# Autodesk Inventor assembly: Pin Header 20x2 TH Pitch 2.54mm v1
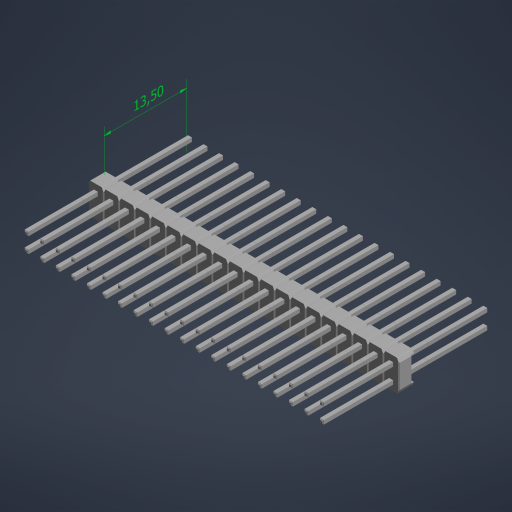
[picture p0: Inventor's stored thumbnail of the model, 512x512]
Saved by Autodesk Inventor 2023 (Build 270158030, 158C)
## iProperties
Created: 2018-05-25
Part Number: Pin Header 20x2 TH Pitch 2.54mm v1
Document SubType Name: Assembly
Designer: Administrator
Title: Pin Header 20x2 TH Pitch 2.54mm v1
Author: Administrator
## Documents named in this file (4)
- C:\Users\norbe\Repozytoria\NormalMapScanner\3D_modeling\construction\parts\external_parts\raspberry_goldpins_2x40\Pin Header 20x2 TH Pitch 2.54mm v1.iam
- C:\Users\norbe\Repozytoria\NormalMapScanner\3D_modeling\construction\parts\external_parts\raspberry_goldpins_2x40\pins.ipt
- C:\Users\norbe\Repozytoria\NormalMapScanner\3D_modeling\construction\parts\external_parts\raspberry_goldpins_2x40\spacers.iam
- C:\Users\norbe\Repozytoria\NormalMapScanner\3D_modeling\construction\parts\external_parts\raspberry_goldpins_2x40\pins_CPY.ipt
## Components (4 placed, 3 different names)
1. pins:1 — Mate:1, Mate:2, Mate:3, Flush:1, Flush:2, Flush:3, Mate:4
2. spacers:1 [sub-assembly] — Mate:1, Mate:2, Mate:3
3. pins_CPY:1 — Flush:1, Flush:2, Flush:3, Mate:4, Flush:4, Flush:5, Mate:5
4. pins_CPY:2 — Flush:4, Flush:5, Mate:5
## Relationships (10: Mate 5, Flush 5)
- Mate:1: pins:1 ↔ spacers:1
- Mate:2: pins:1 ↔ spacers:1
- Mate:3 (-14 mm): pins:1 ↔ spacers:1
- Flush:1: pins:1 ↔ pins_CPY:1
- Flush:2: pins:1 ↔ pins_CPY:1
- Flush:3: pins:1 ↔ pins_CPY:1
- Mate:4 (-1 mm): pins:1 ↔ pins_CPY:1
- Flush:4: pins_CPY:1 ↔ pins_CPY:2
- Flush:5: pins_CPY:1 ↔ pins_CPY:2
- Mate:5 (-2 mm): pins_CPY:1 ↔ pins_CPY:2
